# Autodesk Inventor assembly: TR1 Actuator
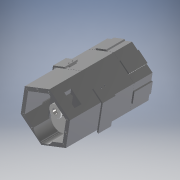
[picture p0: Inventor's stored thumbnail of the model, 180x180]
Saved by Autodesk Inventor 2017 (Build 210142000, 142)
## iProperties
Created: 2018-10-09
Part Number: TR1 Actuator
Document SubType Name: Assembly
Designer: Zach
Author: Zach
## Documents named in this file (23)
- C:\Users\Dell\Documents\GitHub\tr2\Actuator 1.2\Actuator 1.2.iam
- C:\Users\Dell\Documents\GitHub\tr2\Actuator 1.2\TA01.ipt
- C:\Users\Dell\Documents\GitHub\tr2\Actuator 1.2\Arm Actuator\Design Accelerator\Spur Gears2.iam
- C:\Users\Dell\Documents\GitHub\tr2\Actuator 1.2\EMS22XXX-D28-LSX.ipt
- C:\Users\Dell\Documents\GitHub\tr2\Actuator 1.2\12RPM Gear Motor.ipt
- C:\Users\Dell\Documents\GitHub\tr2\Actuator 1.2\Slip Ring.ipt
- C:\Users\Dell\Documents\GitHub\tr2\Actuator 1.2\TA06.ipt
- C:\Users\Dell\Documents\GitHub\tr2\Actuator 1.2\Steel Tubing.ipt
- C:\Users\Dell\Documents\GitHub\tr2\Actuator 1.2\Flange Bearing.ipt
- C:\Users\Dell\Documents\GitHub\tr2\Actuator 1.2\Shaft Collar.ipt
- C:\Users\Dell\Documents\GitHub\tr2\Actuator 1.2\Arm Actuator\Design Accelerator\Spur Gear13.ipt
- C:\Users\Dell\Documents\GitHub\tr2\Actuator 1.2\6mm Mounting Hub, thick.ipt
- C:\Users\Dell\Documents\GitHub\tr2\Actuator 1.2\TA02c.ipt
- C:\Users\Dell\Documents\GitHub\tr2\Actuator 1.2\TA02b.ipt
- C:\Users\Dell\Documents\GitHub\tr2\Actuator 1.2\Bushing.ipt
- C:\Users\Dell\Documents\GitHub\tr2\Actuator 1.2\545340 assembly.iam
- C:\Users\Dell\Documents\GitHub\tr2\Actuator 1.2\TA07.ipt
- C:\Users\Dell\Documents\GitHub\tr2\Actuator 1.2\TA08.ipt
- C:\Users\Dell\Documents\Inventor\Content Center Files\R2017\en-US\BS EN 24017\ISO 4017 - M5 x 35BS EN.ipt
- C:\Users\Dell\Documents\Inventor\Content Center Files\R2017\en-US\BS EN 24017\ISO 4017 - M5 x 40BS EN.ipt
- C:\Users\Dell\Documents\GitHub\tr2\Actuator 1.2\Actuator 1.2\Design Accelerator\Extension Spring1.iam
- C:\Users\Dell\Documents\GitHub\tr2\Actuator 1.2\TA09.ipt
- C:\Users\Dell\Documents\GitHub\tr2\Actuator 1.2\TA09b.ipt
## Components (29 placed, 22 different names)
1. TA01:1 — Mate:130, Mate:161, Mate:164, Mate:165, Mate:166
2. TA06:1 — Mate:34, Mate:35, Mate:82, Mate:83, Mate:129
3. Spur Gears:1 [sub-assembly] — Mate:33, Mate:97, Mate:121, Mate:123, Mate:124, Mate:125, Mate:129
4. 12RPM Gear Motor:1 — Mate:86, Mate:88, Mate:102, Mate:103, Mate:114, Mate:115
5. EMS22XXX-D28-LSX:1 — Mate:118, Mate:126, Angle:1, Mate:134
6. Slip Ring:1 — Mate:33, Mate:34, Mate:35, Mate:83
7. Steel Tubing:1 — Mate:76, Mate:77, Flush:2, Mate:82, Mate:84, Mate:96, Mate:98, Mate:104, Mate:120, Mate:121, Mate:162, Mate:164
8. Flange Bearing:1 — Mate:76, Mate:78, Mate:122
9. Shaft Collar:1 — Mate:77, Mate:78, Flush:2
10. Flange Bearing:2 — Mate:84
11. Spur Gear1:1 — Mate:88, Mate:116
12. 6mm Mounting Hub, thick:1 — Mate:86, Mate:114, Mate:116, Flush:3
13. TA02c:1 — Mate:98, Mate:99, Mate:105, Mate:122, Mate:127, Mate:128, Mate:130, Mate:131, Angle:2, Mate:137, Mate:138, Mate:139, Mate:140, Mate:165, Mate:166
14. TA02b:1 — Mate:96, Mate:97, Mate:99, Mate:102, Mate:103, Mate:115, Mate:126, Angle:1, Mate:131, Mate:132, Mate:133, Mate:134, Mate:141, Mate:150, Mate:151, Mate:152, Mate:153, Mate:158, Mate:159, Mate:160, Mate:163, Mate:167, Mate:168, Mate:169
15. Bushing:1 — Mate:104, Mate:105
16. Spur Gear1:2 — Mate:119
17. 6mm Mounting Hub, thick:2 — Mate:118, Mate:119, Flush:3
18. 545340 assembly:1 [sub-assembly] — Mate:120, Mate:123, Mate:124, Mate:125
19. EMS22XXX-D28-LSX:2 — Mate:127, Mate:128, Angle:2, Mate:135
20. TA07:1 — Mate:132, Mate:133, Mate:136
21. TA08:1 — Mate:135, Mate:136
22. BS EN 24017 - Metric M5 x 35:1 — Mate:139, Mate:140, Mate:149
23. BS EN 24017 - Metric M5 x 35:2 — Mate:137, Mate:138, Mate:146
24. BS EN 24017 - Metric M5 x 40:1 — Mate:141, Mate:147, Mate:163
25. BS EN 24017 - Metric M5 x 40:2 — Mate:148, Mate:152, Mate:153
26. Extension Spring:1 [sub-assembly] — Mate:148, Mate:149, Mate:151
27. Extension Spring:2 [sub-assembly] — Mate:146, Mate:147, Mate:150
28. TA09:2 — Mate:158, Mate:159, Mate:160
29. TA09b:1 — Mate:167, Mate:168, Mate:169
## Relationships (71: Mate 67, Flush 2, Angle 2)
- Mate:33: Spur Gears:1 ↔ Slip Ring:1
- Mate:34: TA06:1 ↔ Slip Ring:1
- Mate:35: TA06:1 ↔ Slip Ring:1
- Mate:76: Steel Tubing:1 ↔ Flange Bearing:1
- Mate:77: Steel Tubing:1 ↔ Shaft Collar:1
- Mate:78: Flange Bearing:1 ↔ Shaft Collar:1
- Flush:2: Steel Tubing:1 ↔ Shaft Collar:1
- Mate:82: TA06:1 ↔ Steel Tubing:1
- Mate:83: TA06:1 ↔ Slip Ring:1
- Mate:84: Steel Tubing:1 ↔ Flange Bearing:2
- Mate:86: 12RPM Gear Motor:1 ↔ 6mm Mounting Hub, thick:1
- Mate:88: 12RPM Gear Motor:1 ↔ Spur Gear1:1
- Mate:96: Steel Tubing:1 ↔ TA02b:1
- Mate:97: Spur Gears:1 ↔ TA02b:1
- Mate:98: Steel Tubing:1 ↔ TA02c:1
- Mate:99: TA02c:1 ↔ TA02b:1
- Mate:102: 12RPM Gear Motor:1 ↔ TA02b:1
- Mate:103: 12RPM Gear Motor:1 ↔ TA02b:1
- Mate:104: Steel Tubing:1 ↔ Bushing:1
- Mate:105: TA02c:1 ↔ Bushing:1
- Mate:114: 12RPM Gear Motor:1 ↔ 6mm Mounting Hub, thick:1
- Mate:115: 12RPM Gear Motor:1 ↔ TA02b:1
- Mate:116: Spur Gear1:1 ↔ 6mm Mounting Hub, thick:1
- [Mate]: Spur Gear1:2 ↔ 6mm Mounting Hub, thick:2
- Mate:118: EMS22XXX-D28-LSX:1 ↔ 6mm Mounting Hub, thick:2
- Mate:119: Spur Gear1:2 ↔ 6mm Mounting Hub, thick:2
- Flush:3: 6mm Mounting Hub, thick:1 ↔ 6mm Mounting Hub, thick:2
- Mate:120: Steel Tubing:1 ↔ 545340 assembly:1
- Mate:121: Spur Gears:1 ↔ Steel Tubing:1
- Mate:122: Flange Bearing:1 ↔ TA02c:1
- Mate:123: Spur Gears:1 ↔ 545340 assembly:1
- Mate:124: Spur Gears:1 ↔ 545340 assembly:1
- Mate:125: Spur Gears:1 ↔ 545340 assembly:1
- Mate:126: EMS22XXX-D28-LSX:1 ↔ TA02b:1
- Angle:1 (0 deg): EMS22XXX-D28-LSX:1 ↔ TA02b:1
- Mate:127: TA02c:1 ↔ EMS22XXX-D28-LSX:2
- Mate:128: TA02c:1 ↔ EMS22XXX-D28-LSX:2
- Mate:129: TA06:1 ↔ Spur Gears:1
- Mate:130: TA01:1 ↔ TA02c:1
- Mate:131: TA02c:1 ↔ TA02b:1
- Angle:2 (0 deg): TA02c:1 ↔ EMS22XXX-D28-LSX:2
- Mate:132: TA02b:1 ↔ TA07:1
- Mate:133: TA02b:1 ↔ TA07:1
- Mate:134: EMS22XXX-D28-LSX:1 ↔ TA02b:1
- Mate:135: EMS22XXX-D28-LSX:2 ↔ TA08:1
- Mate:136: TA07:1 ↔ TA08:1
- Mate:137: TA02c:1 ↔ BS EN 24017 - Metric M5 x 35:2
- Mate:138: TA02c:1 ↔ BS EN 24017 - Metric M5 x 35:2
- Mate:139: TA02c:1 ↔ BS EN 24017 - Metric M5 x 35:1
- Mate:140: TA02c:1 ↔ BS EN 24017 - Metric M5 x 35:1
- Mate:141: TA02b:1 ↔ BS EN 24017 - Metric M5 x 40:1
- Mate:146: BS EN 24017 - Metric M5 x 35:2 ↔ Extension Spring:2
- Mate:147: BS EN 24017 - Metric M5 x 40:1 ↔ Extension Spring:2
- Mate:148: BS EN 24017 - Metric M5 x 40:2 ↔ Extension Spring:1
- Mate:149: BS EN 24017 - Metric M5 x 35:1 ↔ Extension Spring:1
- Mate:150 (10 mm): TA02b:1 ↔ Extension Spring:2
- Mate:151 (10 mm): TA02b:1 ↔ Extension Spring:1
- Mate:152: TA02b:1 ↔ BS EN 24017 - Metric M5 x 40:2
- Mate:153: TA02b:1 ↔ BS EN 24017 - Metric M5 x 40:2
- Mate:158: TA02b:1 ↔ TA09:2
- Mate:159: TA02b:1 ↔ TA09:2
- Mate:160: TA02b:1 ↔ TA09:2
- Mate:161: TA01:1
- Mate:162: Steel Tubing:1
- Mate:163: TA02b:1 ↔ BS EN 24017 - Metric M5 x 40:1
- Mate:164: TA01:1 ↔ Steel Tubing:1
- Mate:165: TA01:1 ↔ TA02c:1
- Mate:166: TA01:1 ↔ TA02c:1
- Mate:167: TA02b:1 ↔ TA09b:1
- Mate:168: TA02b:1 ↔ TA09b:1
- Mate:169: TA02b:1 ↔ TA09b:1
## Named parameters: d140_d139 = 0 mm
